# Autodesk Inventor assembly: Wheel
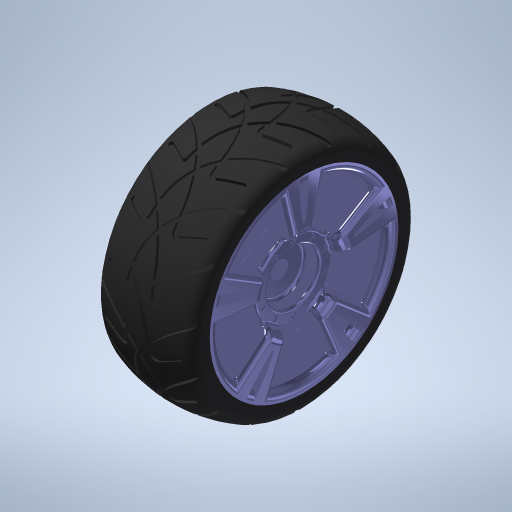
[picture p0: Inventor's stored thumbnail of the model, 512x512]
Saved by Autodesk Inventor 2023.1 (Build 271208000, 208)
## iProperties
Created: 2019-12-04
Part Number: Wheel
Document SubType Name: Assembly
Designer: Jopa
Author: Jopa
## Documents named in this file (3)
- C:\Users\Arzum Naz Doğaner\OneDrive\Masaüstü\HUDSON süspansiyon\Wheel L.iam
- C:\Users\Arzum Naz Doğaner\OneDrive\Masaüstü\HUDSON süspansiyon\Wheel.ipt
- C:\Users\Arzum Naz Doğaner\OneDrive\Masaüstü\HUDSON süspansiyon\Tire.ipt
## Components (2 placed, 2 different names)
1. Wheel:1 — Insert:1, Mate:1
2. Tire:1 — Insert:1, Mate:1
## Relationships (2: Insert 1, Mate 1)
- Insert:1: Wheel:1 ↔ Tire:1
- Mate:1: Wheel:1 ↔ Tire:1
